# Autodesk Inventor assembly: Base
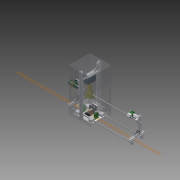
[picture p0: Inventor's stored thumbnail of the model, 180x180]
Saved by Autodesk Inventor 2015 SP1 (Build 190203100, 203)
## iProperties
Created: 2015-02-24
Part Number: Base
Document SubType Name: Assembly
Designer: Andrew
Author: Andrew
## Documents named in this file (31)
- C:\Users\Andrew\Documents\model\Base.iam
- C:\Users\Andrew\Documents\model\Linear Bearing Platform Small.ipt
- C:\Users\Andrew\Documents\model\Base Plate.ipt
- C:\Users\Andrew\Documents\model\NEMA 17 Stepper.ipt
- C:\Users\Andrew\Documents\model\GT2 Pulley.ipt
- C:\Users\Andrew\Documents\model\Stepper Motor Mount.ipt
- C:\Users\Andrew\Documents\model\MainRod.ipt
- C:\Users\Andrew\Documents\model\Linear Rail Shaft Guide.ipt
- C:\Users\Andrew\Documents\model\Belt Tensioner Assy.iam
- C:\Users\Andrew\Documents\model\X-Ray Tube.ipt
- C:\Users\Andrew\Documents\model\Spur Gear.ipt
- C:\Users\Andrew\Documents\model\Worm Gear.ipt
- C:\Users\Andrew\Documents\model\20x20 Slotted Extrusion Arm.ipt
- C:\Users\Andrew\Documents\model\20x20 Slotted Extrusion Tower.ipt
- C:\Users\Andrew\Documents\model\Corner Brace.ipt
- C:\Users\Andrew\Documents\model\Worm Gear Box.ipt
- C:\Users\Andrew\Documents\model\Bearing.ipt
- C:\Users\Andrew\Documents\model\20x20 Slotted Extrusion Stationary Arm.ipt
- C:\Users\Andrew\Documents\model\Clamp Rod.ipt
- C:\Users\Andrew\Documents\model\Rotational Rod.ipt
- C:\Users\Andrew\Documents\model\20x20 Slotted Extrusion Base.ipt
- C:\Users\Andrew\Documents\model\20x20 Slotted Extrusion Source Bracket.ipt
- C:\Users\Andrew\Documents\model\Lead Box Cover.ipt
- C:\Users\Andrew\Documents\model\Lead Box.ipt
- C:\Users\Andrew\Documents\model\Exposure.ipt
- C:\Users\Andrew\Documents\model\Cover.ipt
- C:\Users\Andrew\Documents\model\Tensioning Bracket.ipt
- C:\Users\Andrew\Documents\model\Linear Bearing Platform Adapter Back.ipt
- C:\Users\Andrew\Documents\model\Linear Bearing Platform Adapter.ipt
- C:\Users\Andrew\Documents\model\Part8.ipt
- C:\Users\Andrew\Documents\model\GT2 Belt Cut.ipt
## Components (54 placed, 30 different names)
1. Linear Bearing Platform Small:1 — Flush:5, Mate:7, Flush:9, Flush:11, Flush:12
2. Linear Bearing Platform Small:2 — Flush:4, Flush:5, Flush:6, Mate:6, Angle:2, Flush:8, Flush:10
3. Linear Bearing Platform Small:3 — Flush:4, Mate:8, Flush:8
4. Linear Bearing Platform Small:4 — Flush:6, Mate:1, Mate:9, Angle:3, Flush:9, Flush:13
5. Base Plate:1 — Flush:1, Flush:2, Flush:3, Mate:1, Mate:5, Angle:2, Angle:3, Flush:10, Flush:11, Flush:12, Flush:13, Angle:4, Flush:26, Flush:27, Mate:24, Flush:30, Mate:104, Mate:105, Flush:40, Flush:42, Mate:123, Flush:43, Mate:127
6. NEMA 17 Stepper:1 — Mate:4, Flush:7, Angle:1, Mate:14, Mate:15
7. GT2 Pulley:1 — Mate:4, Flush:7, Mate:22, Mate:112
8. Stepper Motor Mount:1 — Angle:1, Mate:5, Angle:4, Mate:14, Mate:15, Flush:30, Flush:50
9. MainRod:1 — Mate:6, Mate:7, Mate:10, Flush:16, Mate:12, Flush:24
10. MainRod:2 — Mate:8, Mate:9, Mate:11, Flush:16, Mate:13, Flush:23
11. Linear Rail Shaft Guide:1 — Mate:10, Flush:14, Flush:15, Flush:24
12. Linear Rail Shaft Guide:2 — Mate:11, Flush:14, Flush:15, Flush:31, Mate:47, Mate:48
13. Linear Rail Shaft Guide:3 — Mate:12
14. Linear Rail Shaft Guide:4 — Mate:13, Flush:23, Flush:32, Mate:49, Mate:50
15. Belt Tensioner Assy:1 [sub-assembly] — Flush:25, Mate:23, Symmetry:1, Mate:124, Mate:126
16. Belt Tensioner Assy:2 [sub-assembly] — Flush:25, Symmetry:1, Mate:125, Mate:129
17. Base Plate:2 — Flush:26, Flush:27, Mate:24
18. X-Ray Tube:1 — Mate:113, Mate:114, Mate:115, Mate:121, Mate:122
19. Spur Gear:1 — Tangent:1, Mate:44, Mate:46, Angle:5, Mate:87, Mate:99
20. Stepper Motor Mount:2 — Mate:40, Mate:41, Mate:42, Angle:5, Mate:53, Mate:54, Mate:55, Mate:79
21. Worm Gear:1 — Mate:27, Mate:28, Tangent:1, Mate:44, Mate:46, Mate:80
22. NEMA 17 Stepper:2 — Mate:27, Mate:28, Mate:40, Mate:41, Mate:42, Mate:81
23. 20x20 Slotted Extrusion Arm:1 — Flush:31, Mate:47, Mate:48, Mate:52, Flush:34, Mate:66, Mate:68, Mate:70, Mate:72, Mate:100, Mate:138, Angle:8, Mate:140
24. 20x20 Slotted Extrusion Tower:1 — Mate:52, Flush:34, Mate:53, Mate:54, Mate:55, Mate:65, Mate:67, Mate:69, Mate:71
25. 20x20 Slotted Extrusion Arm:2 — Flush:32, Mate:49, Mate:50, Mate:51, Flush:33, Mate:57, Mate:58, Mate:63, Mate:64
26. 20x20 Slotted Extrusion Tower:2 — Mate:51, Flush:33, Mate:59, Mate:60, Mate:61, Mate:62, Angle:7, Mate:88, Mate:89, Mate:90, Flush:35, Flush:36, Mate:92, Mate:95
27. Corner Brace:1 — Mate:69, Mate:70, Mate:71, Mate:72
28. Corner Brace:2 — Mate:65, Mate:66, Mate:67, Mate:68
29. Corner Brace:3 — Mate:57, Mate:58, Mate:59, Mate:60
30. Corner Brace:4 — Mate:61, Mate:62, Mate:63, Mate:64
31. Linear Bearing Platform Small:5 — Mate:86, Angle:6, Mate:87, Mate:91, Mate:93, Mate:130, Mate:131, Mate:132
32. Linear Rail Shaft Guide:5 — Mate:86, Angle:6, Angle:7, Mate:88, Mate:89, Mate:90, Flush:35, Mate:91
33. Worm Gear Box:1 — Mate:79, Mate:80, Mate:81, Mate:82, Mate:84, Flush:37
34. Bearing:1 — Mate:82
35. Bearing:2 — Mate:84
36. 20x20 Slotted Extrusion Stationary Arm:1 — Flush:36, Mate:92, Mate:93, Mate:94, Mate:96, Mate:97, Mate:133
37. Corner Brace:5 — Mate:94, Mate:95, Mate:96, Mate:97
38. Clamp Rod:1 — Mate:98
39. Rotational Rod:1 — Mate:98, Mate:99, Flush:37, Mate:100, Mate:112
40. 20x20 Slotted Extrusion Base:1 — Mate:104, Symmetry:2, Flush:39, Mate:106, Flush:40, Mate:135, Mate:137
41. 20x20 Slotted Extrusion Base:2 — Mate:105, Symmetry:2, Flush:39, Mate:106, Mate:107, Flush:41, Mate:134
42. 20x20 Slotted Extrusion Source Bracket:1 — Mate:107, Flush:41, Mate:119, Mate:120, Mate:136
43. Lead Box Cover:1 — Mate:116, Mate:117, Mate:118
44. Lead Box:1 — Mate:113, Mate:114, Mate:115, Mate:116, Mate:117, Mate:118, Mate:119, Mate:120
45. Exposure:1 — Mate:121, Mate:122
46. Cover:1 — Flush:42, Mate:123, Flush:43
47. Tensioning Bracket:1 — Flush:44, Flush:45, Mate:125, Mate:126, Mate:128, Mate:129
48. Tensioning Bracket:2 — Flush:44, Flush:45, Mate:124, Mate:127, Mate:128
49. Linear Bearing Platform Adapter Back:1 — Flush:46, Flush:47, Mate:133
50. Linear Bearing Platform Adapter:1 — Flush:46, Flush:47, Mate:130, Mate:131, Mate:132
51. Corner Brace:6 — Mate:135, Flush:48, Flush:49, Mate:136, Mate:137
52. Corner Brace:7 — Mate:134, Flush:48, Flush:49
53. Part8:1 — Flush:50
54. GT2 Belt Cut:1 — Mate:138, Angle:8, Mate:140
## Relationships (154: Mate 100, Flush 43, Angle 8, Symmetry 2, Tangent 1)
- Flush:1: Base Plate:1
- Flush:2: Base Plate:1
- Flush:3: Base Plate:1
- Flush:4: Linear Bearing Platform Small:2 ↔ Linear Bearing Platform Small:3
- Flush:5: Linear Bearing Platform Small:1 ↔ Linear Bearing Platform Small:2
- Flush:6: Linear Bearing Platform Small:2 ↔ Linear Bearing Platform Small:4
- Mate:1: Linear Bearing Platform Small:4 ↔ Base Plate:1
- Mate:4: NEMA 17 Stepper:1 ↔ GT2 Pulley:1
- Flush:7: NEMA 17 Stepper:1 ↔ GT2 Pulley:1
- Angle:1 (0 deg): NEMA 17 Stepper:1 ↔ Stepper Motor Mount:1
- Mate:5 (10 mm): Base Plate:1 ↔ Stepper Motor Mount:1
- Mate:6: Linear Bearing Platform Small:2 ↔ MainRod:1
- Mate:7: Linear Bearing Platform Small:1 ↔ MainRod:1
- Mate:8: Linear Bearing Platform Small:3 ↔ MainRod:2
- Mate:9: Linear Bearing Platform Small:4 ↔ MainRod:2
- Mate:10: MainRod:1 ↔ Linear Rail Shaft Guide:1
- Mate:11: MainRod:2 ↔ Linear Rail Shaft Guide:2
- Angle:2 (0 deg): Linear Bearing Platform Small:2 ↔ Base Plate:1
- Angle:3 (0 deg): Linear Bearing Platform Small:4 ↔ Base Plate:1
- Flush:8: Linear Bearing Platform Small:2 ↔ Linear Bearing Platform Small:3
- Flush:9: Linear Bearing Platform Small:1 ↔ Linear Bearing Platform Small:4
- Flush:10 (5 mm): Linear Bearing Platform Small:2 ↔ Base Plate:1
- Flush:11 (5 mm): Linear Bearing Platform Small:1 ↔ Base Plate:1
- Flush:12 (5 mm): Linear Bearing Platform Small:1 ↔ Base Plate:1
- Flush:13 (5 mm): Linear Bearing Platform Small:4 ↔ Base Plate:1
- Flush:14: Linear Rail Shaft Guide:1 ↔ Linear Rail Shaft Guide:2
- Flush:15: Linear Rail Shaft Guide:1 ↔ Linear Rail Shaft Guide:2
- Flush:16: MainRod:1 ↔ MainRod:2
- Angle:4 (180 deg): Base Plate:1 ↔ Stepper Motor Mount:1
- [Flush]: Linear Rail Shaft Guide:3 ↔ Linear Rail Shaft Guide:4
- [Flush]: Linear Rail Shaft Guide:3 ↔ Linear Rail Shaft Guide:4
- Mate:12: MainRod:1 ↔ Linear Rail Shaft Guide:3
- Mate:13: MainRod:2 ↔ Linear Rail Shaft Guide:4
- Mate:14: NEMA 17 Stepper:1 ↔ Stepper Motor Mount:1
- Mate:15: NEMA 17 Stepper:1 ↔ Stepper Motor Mount:1
- Flush:23 (5 mm): MainRod:2 ↔ Linear Rail Shaft Guide:4
- Flush:24 (5 mm): MainRod:1 ↔ Linear Rail Shaft Guide:1
- Mate:22: GT2 Pulley:1
- Flush:25: Belt Tensioner Assy:1 ↔ Belt Tensioner Assy:2
- Mate:23: Belt Tensioner Assy:1
- Flush:26: Base Plate:1 ↔ Base Plate:2
- Flush:27: Base Plate:1 ↔ Base Plate:2
- Mate:24 (65 mm): Base Plate:1 ↔ Base Plate:2
- Mate:27: Worm Gear:1 ↔ NEMA 17 Stepper:2
- Mate:28 (3 mm): Worm Gear:1 ↔ NEMA 17 Stepper:2
- Flush:30: Base Plate:1 ↔ Stepper Motor Mount:1
- Mate:40: Stepper Motor Mount:2 ↔ NEMA 17 Stepper:2
- Mate:41: Stepper Motor Mount:2 ↔ NEMA 17 Stepper:2
- Mate:42: Stepper Motor Mount:2 ↔ NEMA 17 Stepper:2
- Tangent:1: Spur Gear:1 ↔ Worm Gear:1
- Mate:44: Spur Gear:1 ↔ Worm Gear:1
- Mate:46: Spur Gear:1 ↔ Worm Gear:1
- Angle:5 (0 deg): Spur Gear:1 ↔ Stepper Motor Mount:2
- Flush:31: Linear Rail Shaft Guide:2 ↔ 20x20 Slotted Extrusion Arm:1
- Mate:47: Linear Rail Shaft Guide:2 ↔ 20x20 Slotted Extrusion Arm:1
- Mate:48: Linear Rail Shaft Guide:2 ↔ 20x20 Slotted Extrusion Arm:1
- Flush:32: Linear Rail Shaft Guide:4 ↔ 20x20 Slotted Extrusion Arm:2
- Mate:49: Linear Rail Shaft Guide:4 ↔ 20x20 Slotted Extrusion Arm:2
- Mate:50: Linear Rail Shaft Guide:4 ↔ 20x20 Slotted Extrusion Arm:2
- Mate:51: 20x20 Slotted Extrusion Arm:2 ↔ 20x20 Slotted Extrusion Tower:2
- Flush:33: 20x20 Slotted Extrusion Arm:2 ↔ 20x20 Slotted Extrusion Tower:2
- Mate:52: 20x20 Slotted Extrusion Arm:1 ↔ 20x20 Slotted Extrusion Tower:1
- Flush:34: 20x20 Slotted Extrusion Arm:1 ↔ 20x20 Slotted Extrusion Tower:1
- Mate:53: Stepper Motor Mount:2 ↔ 20x20 Slotted Extrusion Tower:1
- Mate:54: Stepper Motor Mount:2 ↔ 20x20 Slotted Extrusion Tower:1
- Mate:55: Stepper Motor Mount:2 ↔ 20x20 Slotted Extrusion Tower:1
- Mate:57: 20x20 Slotted Extrusion Arm:2 ↔ Corner Brace:3
- Mate:58: 20x20 Slotted Extrusion Arm:2 ↔ Corner Brace:3
- Mate:59: 20x20 Slotted Extrusion Tower:2 ↔ Corner Brace:3
- Mate:60: 20x20 Slotted Extrusion Tower:2 ↔ Corner Brace:3
- Mate:61: 20x20 Slotted Extrusion Tower:2 ↔ Corner Brace:4
- Mate:62: 20x20 Slotted Extrusion Tower:2 ↔ Corner Brace:4
- Mate:63: 20x20 Slotted Extrusion Arm:2 ↔ Corner Brace:4
- Mate:64: 20x20 Slotted Extrusion Arm:2 ↔ Corner Brace:4
- Mate:65: 20x20 Slotted Extrusion Tower:1 ↔ Corner Brace:2
- Mate:66: 20x20 Slotted Extrusion Arm:1 ↔ Corner Brace:2
- Mate:67: 20x20 Slotted Extrusion Tower:1 ↔ Corner Brace:2
- Mate:68: 20x20 Slotted Extrusion Arm:1 ↔ Corner Brace:2
- Mate:69: 20x20 Slotted Extrusion Tower:1 ↔ Corner Brace:1
- Mate:70: 20x20 Slotted Extrusion Arm:1 ↔ Corner Brace:1
- Mate:71: 20x20 Slotted Extrusion Tower:1 ↔ Corner Brace:1
- Mate:72: 20x20 Slotted Extrusion Arm:1 ↔ Corner Brace:1
- Mate:79: Stepper Motor Mount:2 ↔ Worm Gear Box:1
- Mate:80: Worm Gear:1 ↔ Worm Gear Box:1
- Mate:81: NEMA 17 Stepper:2 ↔ Worm Gear Box:1
- Mate:82: Worm Gear Box:1 ↔ Bearing:1
- Mate:84: Worm Gear Box:1 ↔ Bearing:2
- Mate:86: Linear Bearing Platform Small:5 ↔ Linear Rail Shaft Guide:5
- Angle:6 (0 deg): Linear Bearing Platform Small:5 ↔ Linear Rail Shaft Guide:5
- Angle:7 (0 deg): 20x20 Slotted Extrusion Tower:2 ↔ Linear Rail Shaft Guide:5
- Mate:87: Spur Gear:1 ↔ Linear Bearing Platform Small:5
- Mate:88: 20x20 Slotted Extrusion Tower:2 ↔ Linear Rail Shaft Guide:5
- Mate:89: 20x20 Slotted Extrusion Tower:2 ↔ Linear Rail Shaft Guide:5
- Mate:90: 20x20 Slotted Extrusion Tower:2 ↔ Linear Rail Shaft Guide:5
- Flush:35 (-5 mm): 20x20 Slotted Extrusion Tower:2 ↔ Linear Rail Shaft Guide:5
- Mate:91 (50 mm): Linear Bearing Platform Small:5 ↔ Linear Rail Shaft Guide:5
- Flush:36: 20x20 Slotted Extrusion Tower:2 ↔ 20x20 Slotted Extrusion Stationary Arm:1
- Mate:92: 20x20 Slotted Extrusion Tower:2 ↔ 20x20 Slotted Extrusion Stationary Arm:1
- Mate:93: Linear Bearing Platform Small:5 ↔ 20x20 Slotted Extrusion Stationary Arm:1
- Mate:94: 20x20 Slotted Extrusion Stationary Arm:1 ↔ Corner Brace:5
- Mate:95: 20x20 Slotted Extrusion Tower:2 ↔ Corner Brace:5
- Mate:96: 20x20 Slotted Extrusion Stationary Arm:1 ↔ Corner Brace:5
- Mate:97: 20x20 Slotted Extrusion Stationary Arm:1 ↔ Corner Brace:5
- Mate:98: Clamp Rod:1 ↔ Rotational Rod:1
- Mate:99: Spur Gear:1 ↔ Rotational Rod:1
- Flush:37 (-5 mm): Worm Gear Box:1 ↔ Rotational Rod:1
- Mate:100: 20x20 Slotted Extrusion Arm:1 ↔ Rotational Rod:1
- Symmetry:1: Belt Tensioner Assy:1 ↔ Belt Tensioner Assy:2
- Mate:104: Base Plate:1 ↔ 20x20 Slotted Extrusion Base:1
- Mate:105: Base Plate:1 ↔ 20x20 Slotted Extrusion Base:2
- Symmetry:2: 20x20 Slotted Extrusion Base:1 ↔ 20x20 Slotted Extrusion Base:2
- Flush:39: 20x20 Slotted Extrusion Base:1 ↔ 20x20 Slotted Extrusion Base:2
- Mate:106 (150 mm): 20x20 Slotted Extrusion Base:1 ↔ 20x20 Slotted Extrusion Base:2
- Flush:40: Base Plate:1 ↔ 20x20 Slotted Extrusion Base:1
- Mate:107: 20x20 Slotted Extrusion Base:2 ↔ 20x20 Slotted Extrusion Source Bracket:1
- Flush:41: 20x20 Slotted Extrusion Base:2 ↔ 20x20 Slotted Extrusion Source Bracket:1
- Mate:112: GT2 Pulley:1 ↔ Rotational Rod:1
- Mate:113: X-Ray Tube:1 ↔ Lead Box:1
- Mate:114: X-Ray Tube:1 ↔ Lead Box:1
- Mate:115: X-Ray Tube:1 ↔ Lead Box:1
- Mate:116: Lead Box Cover:1 ↔ Lead Box:1
- Mate:117: Lead Box Cover:1 ↔ Lead Box:1
- Mate:118: Lead Box Cover:1 ↔ Lead Box:1
- Mate:119: 20x20 Slotted Extrusion Source Bracket:1 ↔ Lead Box:1
- Mate:120: 20x20 Slotted Extrusion Source Bracket:1 ↔ Lead Box:1
- Mate:121: X-Ray Tube:1 ↔ Exposure:1
- Mate:122: X-Ray Tube:1 ↔ Exposure:1
- Flush:42: Base Plate:1 ↔ Cover:1
- Mate:123: Base Plate:1 ↔ Cover:1
- Flush:43: Base Plate:1 ↔ Cover:1
- Flush:44: Tensioning Bracket:1 ↔ Tensioning Bracket:2
- Flush:45: Tensioning Bracket:1 ↔ Tensioning Bracket:2
- Mate:124: Belt Tensioner Assy:1 ↔ Tensioning Bracket:2
- Mate:125: Belt Tensioner Assy:2 ↔ Tensioning Bracket:1
- Mate:126: Belt Tensioner Assy:1 ↔ Tensioning Bracket:1
- Mate:127: Base Plate:1 ↔ Tensioning Bracket:2
- Mate:128 (100 mm): Tensioning Bracket:1 ↔ Tensioning Bracket:2
- Mate:129 (25 mm): Belt Tensioner Assy:2 ↔ Tensioning Bracket:1
- Flush:46: Linear Bearing Platform Adapter Back:1 ↔ Linear Bearing Platform Adapter:1
- Flush:47: Linear Bearing Platform Adapter Back:1 ↔ Linear Bearing Platform Adapter:1
- Mate:130: Linear Bearing Platform Small:5 ↔ Linear Bearing Platform Adapter:1
- Mate:131: Linear Bearing Platform Small:5 ↔ Linear Bearing Platform Adapter:1
- Mate:132: Linear Bearing Platform Small:5 ↔ Linear Bearing Platform Adapter:1
- Mate:133: 20x20 Slotted Extrusion Stationary Arm:1 ↔ Linear Bearing Platform Adapter Back:1
- Mate:134: 20x20 Slotted Extrusion Base:2 ↔ Corner Brace:7
- Mate:135: 20x20 Slotted Extrusion Base:1 ↔ Corner Brace:6
- Flush:48: Corner Brace:6 ↔ Corner Brace:7
- Flush:49: Corner Brace:6 ↔ Corner Brace:7
- Mate:136: 20x20 Slotted Extrusion Source Bracket:1 ↔ Corner Brace:6
- Mate:137: 20x20 Slotted Extrusion Base:1 ↔ Corner Brace:6
- Flush:50 (17.5 mm): Stepper Motor Mount:1 ↔ Part8:1
- Mate:138: 20x20 Slotted Extrusion Arm:1 ↔ GT2 Belt Cut:1
- Angle:8 (0 deg): 20x20 Slotted Extrusion Arm:1 ↔ GT2 Belt Cut:1
- Mate:140: 20x20 Slotted Extrusion Arm:1 ↔ GT2 Belt Cut:1
## Named parameters: d31_d27 = 0 mm, d32_d28 = 0 mm
